# Autodesk Inventor assembly: 装配体2
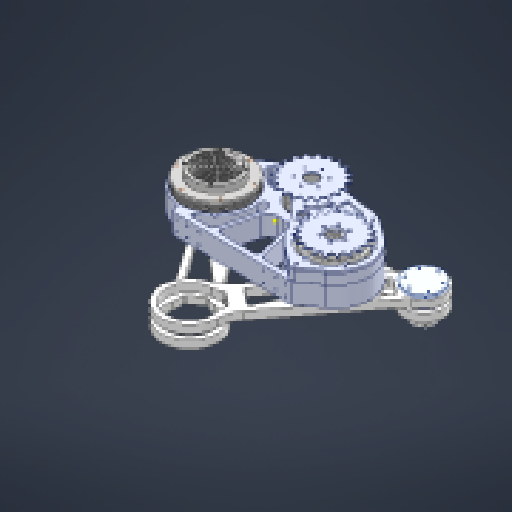
[picture p0: Inventor's stored thumbnail of the model, 512x512]
Saved by Autodesk Inventor 2025 (Build 290162000, 162)
## iProperties
Created: 2025-03-28
Part Number: 装配体2
Document SubType Name: Assembly
Designer: XH
Sending System: SolidWorks 2018
Last Author: Standard
Last Saved: 2025-04-01
代号代码: Assembly.Extension.CustomPropertyManager("").Set("代号",Left(Assembly.GetTitle,InStr(Assembly.GetTitle," ")-1))
名称代码: Assembly.Extension.CustomPropertyManager("").Set("名称",Right(Assembly.GetTitle,Len(Assembly.GetTitle)-InStr(Assembly.GetTitle," ")))
日期: 1800-01-01
名称: 装配体2
Weight: 12.94
版本号: a.1
图样标记S: S
基本计量单位（必填）: 个
Author: XH
## Documents named in this file (22)
- C:\Users\HZD\Desktop\RCInventor\铝件版本\装配体2.iam
- C:\Users\HZD\Desktop\RCInventor\铝件版本\零件6.ipt
- C:\Users\HZD\Desktop\RCInventor\铝件版本\BAR6806.ipt
- C:\Users\HZD\Desktop\RCInventor\铝件版本\零件1.ipt
- C:\Users\HZD\Desktop\RCInventor\铝件版本\61810.ipt
- C:\Users\HZD\Desktop\RCInventor\铝件版本\2.ipt
- C:\Users\HZD\Desktop\RCInventor\铝件版本\零件4.ipt
- C:\Users\HZD\Desktop\RCInventor\铝件版本\31231.ipt
- C:\Users\HZD\Desktop\RCInventor\铝件版本\碗组\标件_碗组总成.iam
- C:\Users\HZD\Desktop\RCInventor\铝件版本\碗组\机加工_碗组连接1.ipt
- C:\Users\HZD\Desktop\RCInventor\铝件版本\碗组\碗组_培林总成.ipt
- C:\Users\HZD\Desktop\RCInventor\铝件版本\碗组\碗组_下底.ipt
- C:\Users\HZD\Desktop\RCInventor\铝件版本\碗组\板材_垫块.ipt
- C:\Users\HZD\Desktop\RCInventor\铝件版本\机加件-髋关节复合固定件.ipt
- C:\Users\HZD\Desktop\RCInventor\铝件版本\碳纤维(cnc)-关节电机端子延展固定.ipt
- C:\Users\HZD\Desktop\RCInventor\铝件版本\dm8009-20240822.iam
- C:\Users\HZD\Desktop\RCInventor\铝件版本\链条\机加件-右关节链轮-20H04A.ipt
- C:\Users\HZD\Desktop\RCInventor\铝件版本\链条\机加件-大腿驱动链轮-20H04A.ipt
- C:\Users\HZD\Desktop\RCInventor\铝件版本\链条\机加件-右关节链轮-20H04A2.ipt
- C:\Users\HZD\Desktop\RCInventor\铝件版本\链条\机加件-大腿驱动链轮-20H04A2.ipt
- C:\Users\HZD\Desktop\RCInventor\铝件版本\链条\标准件-推力轴承52-35-h4.ipt
- C:\Users\HZD\Desktop\RCInventor\铝件版本\链条\碳纤维(cnc)-关节电机端子延展.ipt
## Components (32 placed, 21 different names)
1. 零件6:1 — 配合:8, 配合:44, 配合:45, 配合:47, 配合:53, 配合:79, 配合:86, 配合:88, 配合:100, 配合:101, 配合:103, 配合:104, 配合:105, 配合:106
2. BAR6806:1 — 配合:47, 配合:51, 配合:53
3. 零件1:1 — 配合:45, 配合:46, 配合:48, 配合:49, 配合:51, 配合:56, 配合:59, 配合:81
4. 61810:1 — 配合:44, 配合:58
5. 61810:2 — 配合:46, 配合:59, 配合:73
6. 2:1 — 配合:34, 配合:35, 配合:36, 配合:48, 配合:49, 配合:80, 配合:87
7. 零件4:1 — 配合:5, 配合:8, 配合:9, 配合:63, 配合:64, 配合:88, 配合:101
8. 标件_碗组总成:1 [sub-assembly] — 配合:5, 配合:10, 配合:62, 配合:63
9. 机加工_碗组连接1:1 — 配合:9, 配合:10, 配合:17, 配合:65, 配合:68
10. 碗组_培林总成:1 — 配合:12, 配合:13, 配合:62, 配合:64
11. 碗组_下底:1 — 配合:12, 配合:13
12. 板材_垫块:1 — 配合:17, 配合:66
13. 标件_碗组总成:2 [sub-assembly] — 配合:37, 配合:82, 配合:83, 配合:94, 配合:95
14. 机加工_碗组连接1:2 — 配合:31, 配合:35, 配合:36, 配合:37, 配合:82
15. 碗组_培林总成:2 — 配合:31, 配合:83
16. 碗组_下底:2
17. 板材_垫块:2 — 配合:34
18. 机加件-髋关节复合固定件:1 — 配合:38, 配合:39, 配合:54, 配合:55, 配合:56, 配合:58, 配合:73, 配合:89, 配合:90
19. 碳纤维(cnc)-关节电机端子延展固定:1 — 配合:38, 配合:39, 配合:89, 配合:91, 配合:108, 配合:109
20. dm8009-20240822:1 [sub-assembly] — 配合:90, 配合:91, 配合:98, 配合:99, 配合:107
21. dm8009-20240822:2 [sub-assembly] — 配合:54, 配合:55, 配合:71, 配合:102
22. 31231:2 — 配合:65, 配合:66, 配合:68, 配合:96
23. 机加件-右关节链轮-20H04A:1 — 配合:71, 配合:102, 表面齐平:5
24. 机加件-大腿驱动链轮-20H04A:1 — 配合:78, 表面齐平:3, 配合:80, 配合:81, 表面齐平:5
25. 机加件-右关节链轮-20H04A2:1 — 表面齐平:4, 配合:98, 配合:99
26. 机加件-大腿驱动链轮-20H04A2:1 — 表面齐平:4, 配合:100, 配合:103
27. BAR6806:3 — 配合:78, 表面齐平:3, 配合:79
28. 标准件-推力轴承52-35-h4:1 — 配合:86, 配合:87
29. 31231:3 — 配合:94, 配合:95, 配合:96
30. 标准件-推力轴承52-35-h4:2 — 配合:104, 配合:105
31. 标准件-推力轴承52-35-h4:3 — 配合:106
32. 碳纤维(cnc)-关节电机端子延展:1 — 配合:107, 配合:108, 配合:109
## Relationships (68: Mate 65, Flush 3)
- 配合:5 [Mate]: 零件4:1 ↔ 标件_碗组总成:1
- 配合:8 [Mate]: 零件6:1 ↔ 零件4:1
- 配合:9 [Mate]: 零件4:1 ↔ 机加工_碗组连接1:1
- 配合:10 [Mate]: 标件_碗组总成:1 ↔ 机加工_碗组连接1:1
- 配合:12 [Mate]: 碗组_培林总成:1 ↔ 碗组_下底:1
- 配合:13 [Mate]: 碗组_培林总成:1 ↔ 碗组_下底:1
- 配合:17 [Mate]: 机加工_碗组连接1:1 ↔ 板材_垫块:1
- [Mate]: 碗组_培林总成:2 ↔ 碗组_下底:2
- [Mate]: 碗组_培林总成:2 ↔ 碗组_下底:2
- [Mate]: 机加工_碗组连接1:2 ↔ 板材_垫块:2
- 配合:31 [Mate]: 机加工_碗组连接1:2 ↔ 碗组_培林总成:2
- 配合:34 [Mate]: 2:1 ↔ 板材_垫块:2
- 配合:35 [Mate]: 2:1 ↔ 机加工_碗组连接1:2
- 配合:36 [Mate]: 2:1 ↔ 机加工_碗组连接1:2
- 配合:37 [Mate]: 标件_碗组总成:2 ↔ 机加工_碗组连接1:2
- 配合:38 [Mate]: 机加件-髋关节复合固定件:1 ↔ 碳纤维(cnc)-关节电机端子延展固定:1
- 配合:39 [Mate]: 机加件-髋关节复合固定件:1 ↔ 碳纤维(cnc)-关节电机端子延展固定:1
- 配合:44 [Mate]: 零件6:1 ↔ 61810:1
- 配合:45 [Mate]: 零件6:1 ↔ 零件1:1
- 配合:46 [Mate]: 零件1:1 ↔ 61810:2
- 配合:47 [Mate]: 零件6:1 ↔ BAR6806:1
- 配合:48 [Mate]: 零件1:1 ↔ 2:1
- 配合:49 [Mate]: 零件1:1 ↔ 2:1
- 配合:51 [Mate]: BAR6806:1 ↔ 零件1:1
- 配合:53 [Mate]: 零件6:1 ↔ BAR6806:1
- 配合:54 [Mate]: 机加件-髋关节复合固定件:1 ↔ dm8009-20240822:2
- 配合:55 [Mate]: 机加件-髋关节复合固定件:1 ↔ dm8009-20240822:2
- 配合:56 [Mate]: 零件1:1 ↔ 机加件-髋关节复合固定件:1
- 配合:58 [Mate]: 61810:1 ↔ 机加件-髋关节复合固定件:1
- 配合:59 [Mate]: 零件1:1 ↔ 61810:2
- 配合:62 [Mate]: 标件_碗组总成:1 ↔ 碗组_培林总成:1
- 配合:63 [Mate]: 零件4:1 ↔ 标件_碗组总成:1
- 配合:64 [Mate]: 零件4:1 ↔ 碗组_培林总成:1
- 配合:65 [Mate]: 机加工_碗组连接1:1 ↔ 31231:2
- 配合:66 [Mate]: 板材_垫块:1 ↔ 31231:2
- 配合:68 [Mate]: 机加工_碗组连接1:1 ↔ 31231:2
- 配合:71 [Mate]: dm8009-20240822:2 ↔ 机加件-右关节链轮-20H04A:1
- 配合:73 [Mate]: 61810:2 ↔ 机加件-髋关节复合固定件:1
- 配合:78 [Mate]: 机加件-大腿驱动链轮-20H04A:1 ↔ BAR6806:3
- 表面齐平:3 [Flush]: 机加件-大腿驱动链轮-20H04A:1 ↔ BAR6806:3
- 配合:79 [Mate]: 零件6:1 ↔ BAR6806:3
- 配合:80 [Mate]: 2:1 ↔ 机加件-大腿驱动链轮-20H04A:1
- 配合:81 [Mate]: 零件1:1 ↔ 机加件-大腿驱动链轮-20H04A:1
- 配合:82 [Mate]: 标件_碗组总成:2 ↔ 机加工_碗组连接1:2
- 配合:83 [Mate]: 标件_碗组总成:2 ↔ 碗组_培林总成:2
- 配合:86 [Mate]: 零件6:1 ↔ 标准件-推力轴承52-35-h4:1
- 配合:87 [Mate]: 2:1 ↔ 标准件-推力轴承52-35-h4:1
- 配合:88 [Mate]: 零件6:1 ↔ 零件4:1
- 配合:89 [Mate] (15 mm): 机加件-髋关节复合固定件:1 ↔ 碳纤维(cnc)-关节电机端子延展固定:1
- 配合:90 [Mate]: 机加件-髋关节复合固定件:1 ↔ dm8009-20240822:1
- 配合:91 [Mate]: 碳纤维(cnc)-关节电机端子延展固定:1 ↔ dm8009-20240822:1
- 表面齐平:4 [Flush]: 机加件-右关节链轮-20H04A2:1 ↔ 机加件-大腿驱动链轮-20H04A2:1
- 配合:94 [Mate]: 标件_碗组总成:2 ↔ 31231:3
- 配合:95 [Mate]: 标件_碗组总成:2 ↔ 31231:3
- 配合:96 [Mate]: 31231:2 ↔ 31231:3
- 配合:98 [Mate]: dm8009-20240822:1 ↔ 机加件-右关节链轮-20H04A2:1
- 配合:99 [Mate]: dm8009-20240822:1 ↔ 机加件-右关节链轮-20H04A2:1
- 配合:100 [Mate]: 零件6:1 ↔ 机加件-大腿驱动链轮-20H04A2:1
- 配合:101 [Mate]: 零件6:1 ↔ 零件4:1
- 配合:102 [Mate]: dm8009-20240822:2 ↔ 机加件-右关节链轮-20H04A:1
- 表面齐平:5 [Flush]: 机加件-右关节链轮-20H04A:1 ↔ 机加件-大腿驱动链轮-20H04A:1
- 配合:103 [Mate]: 零件6:1 ↔ 机加件-大腿驱动链轮-20H04A2:1
- 配合:104 [Mate]: 零件6:1 ↔ 标准件-推力轴承52-35-h4:2
- 配合:105 [Mate]: 零件6:1 ↔ 标准件-推力轴承52-35-h4:2
- 配合:106 [Mate]: 零件6:1 ↔ 标准件-推力轴承52-35-h4:3
- 配合:107 [Mate]: dm8009-20240822:1 ↔ 碳纤维(cnc)-关节电机端子延展:1
- 配合:108 [Mate]: 碳纤维(cnc)-关节电机端子延展固定:1 ↔ 碳纤维(cnc)-关节电机端子延展:1
- 配合:109 [Mate]: 碳纤维(cnc)-关节电机端子延展固定:1 ↔ 碳纤维(cnc)-关节电机端子延展:1
## Named parameters: d27_d11 = 0 mm, d28_d12 = 0 mm, d29_d16 = 0 mm
